# Autodesk Inventor assembly: Less but more Complete ROV FRAME!
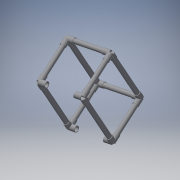
[picture p0: Inventor's stored thumbnail of the model, 180x180]
Saved by Autodesk Inventor 2016 (Build 200138000, 138)
## iProperties
Created: 2017-09-20
Part Number: Less but more Complete ROV FRAME!
Document SubType Name: Assembly
Designer: Student
Author: Student
## Documents named in this file (4)
- C:\Users\Student\Documents\Derek Code and Projects\Autodesk\Less but more Complete ROV FRAME!.iam
- C:\Users\Student\Documents\Derek Code and Projects\CodeBenderCode-master\ROV PVC Pipes\Frame Part 1 (1).ipt
- C:\Users\Student\Documents\Derek Code and Projects\CodeBenderCode-master\ROV PVC Pipes\Frame Part 1.5 (1).ipt
- C:\Users\Student\Documents\Derek Code and Projects\CodeBenderCode-master\ROV PVC Pipes\pvc 1in 3 way elbow.ipt
## Components (18 placed, 3 different names)
1. Frame Part 1 (1):1 — Mate:22, Mate:23, Mate:29
2. Frame Part 1 (1):2 — Mate:9, Mate:10, Mate:11, Mate:12
3. Frame Part 1 (1):3 — Mate:20, Mate:21, Mate:28, Mate:30
4. Frame Part 1 (1):4 — Mate:18, Mate:19, Mate:24, Mate:27
5. Frame Part 1 (1):7 — Mate:16, Mate:17, Mate:25
6. Frame Part 1 (1):8 — Mate:1, Mate:2, Mate:3, Mate:4
7. Frame Part 1.5 (1):1 — Mate:13, Mate:14, Mate:15
8. Frame Part 1.5 (1):2 — Mate:32, Mate:33
9. Frame Part 1.5 (1):3 — Mate:5, Mate:6, Mate:7, Mate:8
10. Frame Part 1.5 (1):4 — Mate:34, Mate:35
11. pvc 1in 3 way elbow:1 — Mate:3, Mate:4, Mate:5, Mate:6, Mate:22, Mate:23
12. pvc 1in 3 way elbow:2 — Mate:7, Mate:8, Mate:9, Mate:10, Mate:18, Mate:19
13. pvc 1in 3 way elbow:3 — Mate:11, Mate:12, Mate:13, Mate:14, Mate:16, Mate:17
14. pvc 1in 3 way elbow:4 — Mate:1, Mate:2, Mate:15, Mate:20, Mate:21
15. pvc 1in 3 way elbow:5 — Mate:25, Mate:26, Mate:32, Mate:33
16. pvc 1in 3 way elbow:6 — Mate:24, Mate:26, Mate:27, Mate:34
17. pvc 1in 3 way elbow:7 — Mate:29, Mate:31, Mate:35
18. pvc 1in 3 way elbow:8 — Mate:28, Mate:30, Mate:31
## Relationships (35: Mate 35)
- Mate:1: Frame Part 1 (1):8 ↔ pvc 1in 3 way elbow:4
- Mate:2: Frame Part 1 (1):8 ↔ pvc 1in 3 way elbow:4
- Mate:3: Frame Part 1 (1):8 ↔ pvc 1in 3 way elbow:1
- Mate:4: Frame Part 1 (1):8 ↔ pvc 1in 3 way elbow:1
- Mate:5: Frame Part 1.5 (1):3 ↔ pvc 1in 3 way elbow:1
- Mate:6: Frame Part 1.5 (1):3 ↔ pvc 1in 3 way elbow:1
- Mate:7: Frame Part 1.5 (1):3 ↔ pvc 1in 3 way elbow:2
- Mate:8: Frame Part 1.5 (1):3 ↔ pvc 1in 3 way elbow:2
- Mate:9: Frame Part 1 (1):2 ↔ pvc 1in 3 way elbow:2
- Mate:10: Frame Part 1 (1):2 ↔ pvc 1in 3 way elbow:2
- Mate:11: Frame Part 1 (1):2 ↔ pvc 1in 3 way elbow:3
- Mate:12: Frame Part 1 (1):2 ↔ pvc 1in 3 way elbow:3
- Mate:13: Frame Part 1.5 (1):1 ↔ pvc 1in 3 way elbow:3
- Mate:14: Frame Part 1.5 (1):1 ↔ pvc 1in 3 way elbow:3
- Mate:15: Frame Part 1.5 (1):1 ↔ pvc 1in 3 way elbow:4
- Mate:16: Frame Part 1 (1):7 ↔ pvc 1in 3 way elbow:3
- Mate:17: Frame Part 1 (1):7 ↔ pvc 1in 3 way elbow:3
- Mate:18: Frame Part 1 (1):4 ↔ pvc 1in 3 way elbow:2
- Mate:19: Frame Part 1 (1):4 ↔ pvc 1in 3 way elbow:2
- Mate:20: Frame Part 1 (1):3 ↔ pvc 1in 3 way elbow:4
- Mate:21: Frame Part 1 (1):3 ↔ pvc 1in 3 way elbow:4
- Mate:22: Frame Part 1 (1):1 ↔ pvc 1in 3 way elbow:1
- Mate:23: Frame Part 1 (1):1 ↔ pvc 1in 3 way elbow:1
- Mate:24: Frame Part 1 (1):4 ↔ pvc 1in 3 way elbow:6
- Mate:25: Frame Part 1 (1):7 ↔ pvc 1in 3 way elbow:5
- Mate:26: pvc 1in 3 way elbow:5 ↔ pvc 1in 3 way elbow:6
- Mate:27: Frame Part 1 (1):4 ↔ pvc 1in 3 way elbow:6
- Mate:28: Frame Part 1 (1):3 ↔ pvc 1in 3 way elbow:8
- Mate:29: Frame Part 1 (1):1 ↔ pvc 1in 3 way elbow:7
- Mate:30: Frame Part 1 (1):3 ↔ pvc 1in 3 way elbow:8
- Mate:31: pvc 1in 3 way elbow:7 ↔ pvc 1in 3 way elbow:8
- Mate:32: Frame Part 1.5 (1):2 ↔ pvc 1in 3 way elbow:5
- Mate:33: Frame Part 1.5 (1):2 ↔ pvc 1in 3 way elbow:5
- Mate:34: Frame Part 1.5 (1):4 ↔ pvc 1in 3 way elbow:6
- Mate:35: Frame Part 1.5 (1):4 ↔ pvc 1in 3 way elbow:7
